# Autodesk Inventor assembly: pickGuardAssembly01
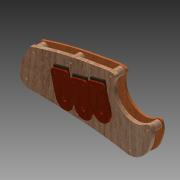
[picture p0: Inventor's stored thumbnail of the model, 180x180]
Saved by Autodesk Inventor 2013 (Build 170138000, 138)
## iProperties
Created: 2014-04-23
Part Number: pickGuardAssembly01
Document SubType Name: Assembly
Designer: Nano
Author: Nano
## Documents named in this file (6)
- C:\Users\Nano\Documents\InventorByron\InventorMasterProject\gyroPhone01\pickGuardAssembly02.iam
- C:\Users\Nano\Documents\InventorByron\InventorMasterProject\gyroPhone01\fingerBase01.ipt
- C:\Users\Nano\Documents\InventorByron\InventorMasterProject\gyroPhone01\pickGuard04.ipt
- C:\Users\Nano\Documents\InventorByron\InventorMasterProject\gyroPhone01\spacerBlock01.ipt
- C:\Users\Nano\Documents\InventorByron\InventorMasterProject\gyroPhone01\mountingBase02.ipt
- C:\Users\Nano\Documents\InventorByron\InventorMasterProject\gyroPhone01\offsetWasher01.ipt
## Components (22 placed, 5 different names)
1. pickGuard04:1 — Flush:1, Flush:2, Mate:1, Mate:2, Mate:3, Mate:4, Mate:5, Mate:6, Flush:3, Flush:4, Mate:7, Mate:8, Mate:10, Mate:11, Mate:12, Mate:13, Mate:14, Mate:15
2. fingerBase01:1 — Flush:1, Flush:2
3. fingerBase01:2 — Mate:1, Mate:2, Mate:3, Mate:9
4. fingerBase01:3 — Mate:4, Mate:5, Mate:6
5. spacerBlock01:1 — Flush:3, Flush:4
6. spacerBlock01:2 — Mate:7, Mate:8, Mate:9
7. spacerBlock01:3 — Mate:10, Mate:11, Mate:12
8. mountingBase02:1 — Mate:13, Mate:14, Mate:15, Flush:5, Flush:6, Mate:18, Mate:19, Mate:22, Mate:23, Mate:26, Mate:27, Mate:30, Mate:31, Mate:34, Mate:35, Mate:38, Mate:39
9. offsetWasher01:1 — Flush:5, Flush:6, Mate:16, Mate:17
10. offsetWasher01:2 — Mate:16, Mate:17
11. offsetWasher01:3 — Mate:30, Mate:31, Mate:32, Mate:33
12. offsetWasher01:4 — Mate:32, Mate:33
13. offsetWasher01:5 — Mate:40, Mate:41
14. offsetWasher01:6 — Mate:20, Mate:21
15. offsetWasher01:7 — Mate:18, Mate:19, Mate:20, Mate:21
16. offsetWasher01:8 — Mate:38, Mate:39, Mate:40, Mate:41
17. offsetWasher01:9 — Mate:36, Mate:37
18. offsetWasher01:10 — Mate:34, Mate:35, Mate:36, Mate:37
19. offsetWasher01:11 — Mate:28, Mate:29
20. offsetWasher01:12 — Mate:26, Mate:27, Mate:28, Mate:29
21. offsetWasher01:13 — Mate:24, Mate:25
22. offsetWasher01:14 — Mate:22, Mate:23, Mate:24, Mate:25
## Relationships (47: Mate 41, Flush 6)
- Flush:1: pickGuard04:1 ↔ fingerBase01:1
- Flush:2: pickGuard04:1 ↔ fingerBase01:1
- Mate:1: pickGuard04:1 ↔ fingerBase01:2
- Mate:2: pickGuard04:1 ↔ fingerBase01:2
- Mate:3: pickGuard04:1 ↔ fingerBase01:2
- Mate:4: pickGuard04:1 ↔ fingerBase01:3
- Mate:5: pickGuard04:1 ↔ fingerBase01:3
- Mate:6: pickGuard04:1 ↔ fingerBase01:3
- Flush:3: pickGuard04:1 ↔ spacerBlock01:1
- Flush:4: pickGuard04:1 ↔ spacerBlock01:1
- Mate:7: pickGuard04:1 ↔ spacerBlock01:2
- Mate:8: pickGuard04:1 ↔ spacerBlock01:2
- Mate:9: fingerBase01:2 ↔ spacerBlock01:2
- Mate:10: pickGuard04:1 ↔ spacerBlock01:3
- Mate:11: pickGuard04:1 ↔ spacerBlock01:3
- Mate:12: pickGuard04:1 ↔ spacerBlock01:3
- Mate:13 (12.7 mm): pickGuard04:1 ↔ mountingBase02:1
- Mate:14: pickGuard04:1 ↔ mountingBase02:1
- Mate:15: pickGuard04:1 ↔ mountingBase02:1
- Flush:5: mountingBase02:1 ↔ offsetWasher01:1
- Flush:6: mountingBase02:1 ↔ offsetWasher01:1
- Mate:16: offsetWasher01:1 ↔ offsetWasher01:2
- Mate:17: offsetWasher01:1 ↔ offsetWasher01:2
- Mate:18: mountingBase02:1 ↔ offsetWasher01:7
- Mate:19: mountingBase02:1 ↔ offsetWasher01:7
- Mate:20: offsetWasher01:6 ↔ offsetWasher01:7
- Mate:21: offsetWasher01:6 ↔ offsetWasher01:7
- Mate:22: mountingBase02:1 ↔ offsetWasher01:14
- Mate:23: mountingBase02:1 ↔ offsetWasher01:14
- Mate:24: offsetWasher01:13 ↔ offsetWasher01:14
- Mate:25: offsetWasher01:13 ↔ offsetWasher01:14
- Mate:26: mountingBase02:1 ↔ offsetWasher01:12
- Mate:27: mountingBase02:1 ↔ offsetWasher01:12
- Mate:28: offsetWasher01:11 ↔ offsetWasher01:12
- Mate:29: offsetWasher01:11 ↔ offsetWasher01:12
- Mate:30: mountingBase02:1 ↔ offsetWasher01:3
- Mate:31: mountingBase02:1 ↔ offsetWasher01:3
- Mate:32: offsetWasher01:3 ↔ offsetWasher01:4
- Mate:33: offsetWasher01:3 ↔ offsetWasher01:4
- Mate:34: mountingBase02:1 ↔ offsetWasher01:10
- Mate:35: mountingBase02:1 ↔ offsetWasher01:10
- Mate:36: offsetWasher01:9 ↔ offsetWasher01:10
- Mate:37: offsetWasher01:9 ↔ offsetWasher01:10
- Mate:38: mountingBase02:1 ↔ offsetWasher01:8
- Mate:39: mountingBase02:1 ↔ offsetWasher01:8
- Mate:40: offsetWasher01:5 ↔ offsetWasher01:8
- Mate:41: offsetWasher01:5 ↔ offsetWasher01:8
